# Autodesk Inventor assembly: WireSlottedHoles
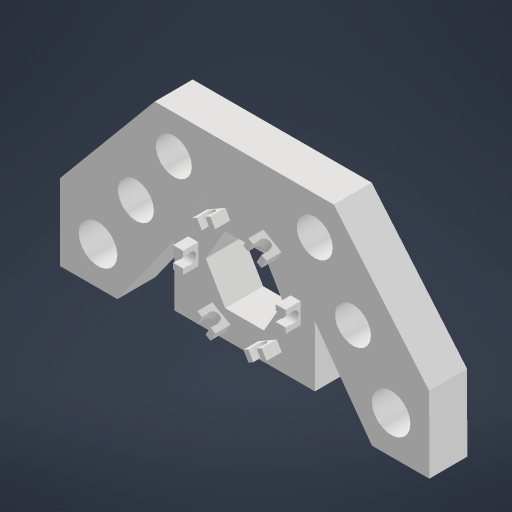
[picture p0: Inventor's stored thumbnail of the model, 512x512]
Saved by Autodesk Inventor 2024.1 (Build 281209000, 209)
## iProperties
Created: 2023-08-21
Part Number: WireSlottedHoles
Document SubType Name: Assembly
Designer: Eleanor
Author: Eleanor
## Documents named in this file (3)
- C:\Users\Eleanor\Documents\Inventor\4.5MM Electromanetic Rifle\WireSlottedHoles.iam
- C:\Users\Eleanor\Documents\Inventor\4.5MM Electromanetic Rifle\WireSlot.ipt
- C:\Users\Eleanor\Documents\Inventor\4.5MM Electromanetic Rifle\WireGuideBoltHols.ipt
## Components (7 placed, 2 different names)
1. WireGuideBoltHols:1 — Mate:4, Mate:5, Angle:1, Mate:7, Mate:8, Mate:9, Mate:10, Mate:11, Mate:12, Angle:2
2. WireSlot:1 — Mate:4, Mate:6
3. WireSlot:2
4. WireSlot:3
5. WireSlot:4
6. WireSlot:5
7. WireSlot:6
## Component patterns: (6 elements, first: WireSlot:1)
## Relationships (14: Mate 12, Angle 2)
- Mate:4: WireGuideBoltHols:1 ↔ WireSlot:1
- Mate:5: WireGuideBoltHols:1
- Angle:1 (0 deg): WireGuideBoltHols:1
- Mate:6: WireSlot:1
- Mate:7: WireGuideBoltHols:1
- Mate:8: WireGuideBoltHols:1
- Mate:9: WireGuideBoltHols:1
- Mate:10: WireGuideBoltHols:1
- Mate:11: WireGuideBoltHols:1
- Mate:12: WireGuideBoltHols:1
- Mate:13
- Mate:14
- Mate:15
- Angle:2 (90 deg): WireGuideBoltHols:1
